# Autodesk Inventor assembly: Full_Rail_Assembly
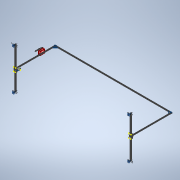
[picture p0: Inventor's stored thumbnail of the model, 180x180]
Saved by Autodesk Inventor 2021 (Build 250183000, 183)
## iProperties
Created: 2021-05-05
Part Number: Full_Rail_Assembly
Document SubType Name: Assembly
Designer: Jorian Brusind
Author: Jorian Brusind
## Documents named in this file (4)
- C:\Users\Jorian Brusind\Documents\GitHub\PersonalProjects\HyperRail\Inventor Files\Full_Rail_Assembly.iam
- C:\Users\Jorian Brusind\Documents\GitHub\PersonalProjects\HyperRail\Inventor Files\Ebox_assy.iam
- C:\Users\Jorian Brusind\Documents\GitHub\PersonalProjects\HyperRail\Inventor Files\Rail_AssemblyV2_0.iam
- C:\Users\Jorian Brusind\Documents\GitHub\PersonalProjects\HyperRail\Inventor Files\Top_Rail_Section.iam
## Components (6 placed, 3 different names)
1. Ebox_assy:1 [sub-assembly] — Mate:8, Flush:9, Flush:10
2. Top_Rail_Section:1 [sub-assembly] — Mate:6, Flush:6, Flush:7, Flush:8, Mate:7, Flush:9
3. Top_Rail_Section:2 [sub-assembly] — Mate:5, Flush:4, Flush:5, Mate:6, Flush:6, Flush:7
4. Top_Rail_Section:3 [sub-assembly] — Flush:3, Mate:3, Mate:4, Mate:5, Flush:4, Flush:5
5. Rail_AssemblyV2_0:1 [sub-assembly] — Flush:1, Flush:8, Mate:7, Mate:8, Flush:10
6. Rail_AssemblyV2_0:2 [sub-assembly] — Flush:1, Flush:2, Mate:1, Mate:2, Flush:3, Mate:3, Mate:4
## Relationships (18: Flush 10, Mate 8)
- Flush:1: Rail_AssemblyV2_0:1 ↔ Rail_AssemblyV2_0:2
- Flush:2: Rail_AssemblyV2_0:2
- Mate:1: Rail_AssemblyV2_0:2
- Mate:2: Rail_AssemblyV2_0:2
- Flush:3: Top_Rail_Section:3 ↔ Rail_AssemblyV2_0:2
- Mate:3: Top_Rail_Section:3 ↔ Rail_AssemblyV2_0:2
- Mate:4: Top_Rail_Section:3 ↔ Rail_AssemblyV2_0:2
- Mate:5: Top_Rail_Section:2 ↔ Top_Rail_Section:3
- Flush:4: Top_Rail_Section:2 ↔ Top_Rail_Section:3
- Flush:5: Top_Rail_Section:2 ↔ Top_Rail_Section:3
- Mate:6: Top_Rail_Section:1 ↔ Top_Rail_Section:2
- Flush:6: Top_Rail_Section:1 ↔ Top_Rail_Section:2
- Flush:7: Top_Rail_Section:1 ↔ Top_Rail_Section:2
- Flush:8: Top_Rail_Section:1 ↔ Rail_AssemblyV2_0:1
- Mate:7: Top_Rail_Section:1 ↔ Rail_AssemblyV2_0:1
- Mate:8: Ebox_assy:1 ↔ Rail_AssemblyV2_0:1
- Flush:9 (600 mm): Ebox_assy:1 ↔ Top_Rail_Section:1
- Flush:10 (-25 mm): Ebox_assy:1 ↔ Rail_AssemblyV2_0:1
